# Autodesk Inventor assembly: 559278 DSNU-20-200-PPS-A---(0)
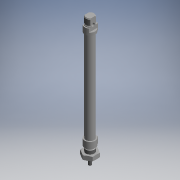
[picture p0: Inventor's stored thumbnail of the model, 180x180]
Saved by Autodesk Inventor 2017.3 (Build 213256000, 256)
## iProperties
Category: PARTsolutions
Company: FESTO
Part Number: 559278 DSNU-20-200-PPS-A---(0)
Catalog Web Link: www.cadenas.de
Description: DSNU-Round cylinder
Vendor: FESTO
Document SubType Name: Assembly
Designer: partserver
Manufacturer: FESTO
Mass: 330.8 g
Surface Area: 491.997 cm^2
Volume: 66.8332 cm^3
Density: 4.94964 g/cm^3
Title: 559278 DSNU-20-200-PPS-A
Author: Cadenas PARTsolutions
Comments: Round cylinder
PSOL_IDENT_0: {ATYP=ASSISTANT},{DATA=script=$CADENAS_DATA/23d-libs/festo/webfesto.vbb&M_FAMILY=DSNU&M_GROUP=01&M_P
PSOL_IDENT_1: ARTNO=559278&IDCODE1=DSNU-20-200-PPS-A&IDCODE2=&customer_number_cns=&MATES=1&LOD=HI&LOCKERP=0&SINGLE
PSOL_IDENT_2: PART=1}
NB: 559278 DSNU-20-200-PPS-A---(0)
NN: DSNU
NT: Round cylinder
NBSYN: $NB1.---($HUBST.)
LINA: 559278 DSNU-20-200-PPS-A
CATALOG: Festo
OFFICIAL_STANDARD_NUMBERS: ISO 6432
TNR: 559278
TYP: DSNU-20
KDM: 20
HUB: 200
HUBST: 0
DA: PPS
PE: A
KS: -
A1: 25
A2: 110
A3: 8
A4: 47
AB: 22
AM: 20
B: 22
BB: 3
BE: M22x1,5
BS: 5.5
B1: 40
B2: 0
B3: 0
B4: 0
B5: 22.4
B6: 10
B7: 0
CD: 8
D: 27
D1: 22
D2: 8
D3: 21.3
D4: 7
D5: 21.7
D6: 0
D7: 0
EE: G1/8
EW: 16
F: 31
FF: M5
F1: 0
H: 28
H1: 0
KK: M8
K1: M4
K2: 0
KV: 32
KW: 11
KV2: 0
KW2: 0
L: 12
LH: 7.5
LK: 14.5
L1: 312
L2: 268
L3: 8.2
L4: 20
L5: 18
L6: 44
L7: 24
L8: 16
L9: 29
L13: 116
ST: 5.5
SW: 7
T: 12
WH: 24
X: 2
XC: 295
CNSMASSEXACT: 0.3308
SUPPLIER: FESTO
ARTICLENO: 559278 DSNU-20-200-PPS-A---(0)
BOMINFO: 559278 DSNU-20-200-PPS-A
CREATOR: CADENAS GmbH
## Documents named in this file (4)
- e:\temp\worker_7\temp\exporttempdir_1052_239_IDCWM\format_0\559278 DSNU-20-200-PPS-A---(0).iam
- e:\temp\worker_7\temp\exporttempdir_1052_239_IDCWM\format_0\559278 DSNU-20-200-PPS---(A----0-ZR).ipt
- e:\temp\worker_7\temp\exporttempdir_1052_239_IDCWM\format_0\DIN-439-B - M22x1_5(F).ipt
- e:\temp\worker_7\temp\exporttempdir_1052_239_IDCWM\format_0\559278 DSNU-20-200-PPS---(A---00--0-KS).ipt
## Components (3 placed, 3 different names)
1. 559278 DSNU-20-200-PPS---(A----0-ZR):1 — NUT_XY@1 <-> 2CYL_XY@2, NUT_Z@1 <-> 2CYL_Z@2, NUT_YZ@1 <-> 2CYL_YZ@2
2. DIN-439-B - M22x1_5(F):1 — NUT_XY@1 <-> 2CYL_XY@2, NUT_Z@1 <-> 2CYL_Z@2, NUT_YZ@1 <-> 2CYL_YZ@2
3. 559278 DSNU-20-200-PPS---(A---00--0-KS):1
## Relationships (3: Mate 2, Angle 1)
- NUT_XY@1 <-> 2CYL_XY@2 [Mate] (-5.5 mm): 559278 DSNU-20-200-PPS---(A----0-ZR):1 ↔ DIN-439-B - M22x1_5(F):1
- NUT_Z@1 <-> 2CYL_Z@2 [Mate]: 559278 DSNU-20-200-PPS---(A----0-ZR):1 ↔ DIN-439-B - M22x1_5(F):1
- NUT_YZ@1 <-> 2CYL_YZ@2 [Angle] (0 deg): 559278 DSNU-20-200-PPS---(A----0-ZR):1 ↔ DIN-439-B - M22x1_5(F):1
